# Autodesk Inventor assembly: Ensamble_2
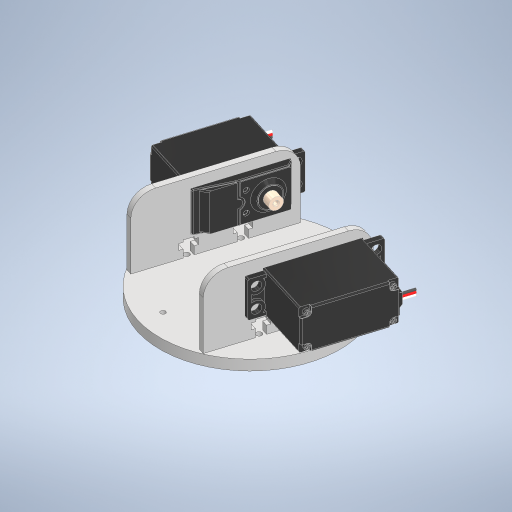
[picture p0: Inventor's stored thumbnail of the model, 512x512]
Saved by Autodesk Inventor 2023 (Build 270158000, 158)
## iProperties
Created: 2024-09-27
Part Number: Ensamble_2
Document SubType Name: Assembly
Designer: sebas
Author: sebas
## Documents named in this file (3)
- C:\Users\sebas\OneDrive\Documentos\ILLERO_MODELADO_ROBOT\Ensamble_2.iam
- C:\Users\sebas\OneDrive\Documentos\ILLERO_MODELADO_ROBOT\Pieza_base_2.ipt
- C:\Users\sebas\OneDrive\Documentos\ILLERO_MODELADO_ROBOT\User Library-Subasa Servo S3003.ipt
## Components (3 placed, 2 different names)
1. Pieza_base_2:1 — Coincidencia:19, Coincidencia:20, Coincidencia:21, Coincidencia:22, Coincidencia:23, Coincidencia:24
2. User Library-Subasa Servo S3003:1 — Coincidencia:19, Coincidencia:20, Coincidencia:21
3. User Library-Subasa Servo S3003:5 — Coincidencia:22, Coincidencia:23, Coincidencia:24
## Relationships (6: Mate 6)
- Coincidencia:19 [Mate]: Pieza_base_2:1 ↔ User Library-Subasa Servo S3003:1
- Coincidencia:20 [Mate]: Pieza_base_2:1 ↔ User Library-Subasa Servo S3003:1
- Coincidencia:21 [Mate]: Pieza_base_2:1 ↔ User Library-Subasa Servo S3003:1
- Coincidencia:22 [Mate]: Pieza_base_2:1 ↔ User Library-Subasa Servo S3003:5
- Coincidencia:23 [Mate]: Pieza_base_2:1 ↔ User Library-Subasa Servo S3003:5
- Coincidencia:24 [Mate]: Pieza_base_2:1 ↔ User Library-Subasa Servo S3003:5
